# Autodesk Inventor assembly: stepper_motor
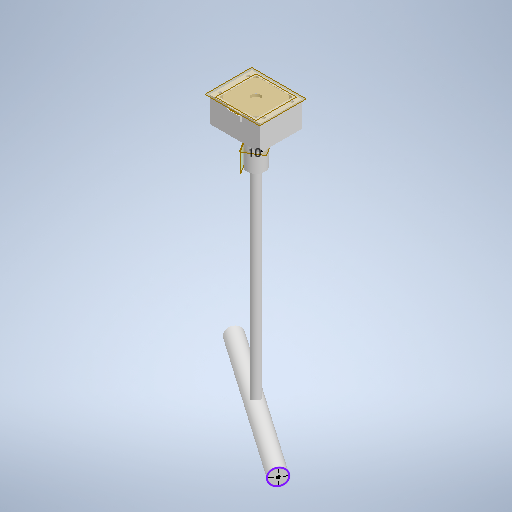
[picture p0: Inventor's stored thumbnail of the model, 512x512]
Saved by Autodesk Inventor 2025.1 (Build 291241000, 241)
## iProperties
Created: 2024-11-23
Part Number: stepper_motor
Document SubType Name: Assembly
Designer: dell
Author: dell
## Documents named in this file (5)
- D:\creap\Tonbo.iam
- D:\creap\joint.ipt
- D:\creap\Tonbo.ipt
- D:\creap\stepper_motor.ipt
- D:\creap\motor_case2.ipt
## Components (4 placed, 4 different names)
1. joint:1 — 回転:1, 挿入:5
2. Tonbo:1 — 挿入:5
3. stepper_motor:1 — 挿入:3, 挿入:4, 回転:1
4. motor_case2:1 — 挿入:3, 挿入:4
## Relationships (4: Insert 3, RevoluteJoint 1)
- 挿入:3 [Insert]: stepper_motor:1 ↔ motor_case2:1
- 挿入:4 [Insert]: stepper_motor:1 ↔ motor_case2:1
- 回転:1 [RevoluteJoint]: joint:1 ↔ stepper_motor:1
- 挿入:5 [Insert]: joint:1 ↔ Tonbo:1
